# Autodesk Inventor assembly: PIEZA DERIVADA + MATERIAL MOLDE 1
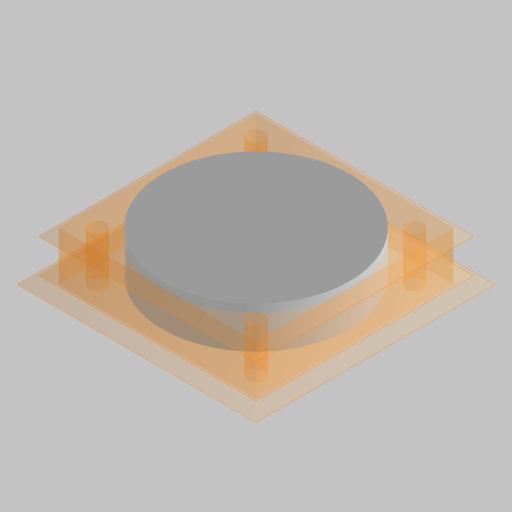
[picture p0: Inventor's stored thumbnail of the model, 512x512]
Saved by Autodesk Inventor 2024 (Build 280153000, 153)
## iProperties
Created: 2023-02-13
Part Number: PIEZA DERIVADA + MATERIAL MOLDE 1
Document SubType Name: Assembly
Designer: rodar
Author: rodar
## Documents named in this file (3)
- G:\Unidades compartidas\Cursos de Ingeniería Mecánica UVG\Cursos IMXXX\IM3027 Introducción a Diseño y Manufactura CAD CAM\Clases - 2do semestre 2023\S7C1 - INVENTOR CAM\3 - PIEZA DERIVADA + MATERIAL MOLDE 1.iam
- G:\Unidades compartidas\Cursos de Ingeniería Mecánica UVG\Cursos IMXXX\IM3027 Introducción a Diseño y Manufactura CAD CAM\Clases - 2do semestre 2023\S7C1 - INVENTOR CAM\2 - PIEZA DERIVADA.ipt
- G:\Unidades compartidas\Cursos de Ingeniería Mecánica UVG\Cursos IMXXX\IM3027 Introducción a Diseño y Manufactura CAD CAM\Clases - 2do semestre 2023\S7C1 - INVENTOR CAM\3 - MATERIAL MOLDE 1.ipt
## Components (2 placed, 2 different names)
1. 2 - PIEZA DERIVADA:1
2. 3 - MATERIAL MOLDE 1:1 — Flush:1
## Relationships (1: Flush 1)
- Flush:1: 3 - MATERIAL MOLDE 1:1
